# Autodesk Inventor assembly: FRC Fixed Field 2018_sldasm
(part 2 of 2)
- C:\Users\CAD\Documents\GitHub\FIRST Power Up Field CAD\Body_1165_sldprt.ipt
- C:\Users\CAD\Documents\GitHub\FIRST Power Up Field CAD\Body_1166_sldprt.ipt
- C:\Users\CAD\Documents\GitHub\FIRST Power Up Field CAD\Body_1167_sldprt.ipt
- C:\Users\CAD\Documents\GitHub\FIRST Power Up Field CAD\Body_1168_sldprt.ipt
- C:\Users\CAD\Documents\GitHub\FIRST Power Up Field CAD\Body_1169_sldprt.ipt
- C:\Users\CAD\Documents\GitHub\FIRST Power Up Field CAD\Body_1170_sldprt.ipt
- C:\Users\CAD\Documents\GitHub\FIRST Power Up Field CAD\Body_1171_sldprt.ipt
- C:\Users\CAD\Documents\GitHub\FIRST Power Up Field CAD\Body_1172_sldprt.ipt
- C:\Users\CAD\Documents\GitHub\FIRST Power Up Field CAD\Body_1173_sldprt.ipt
- C:\Users\CAD\Documents\GitHub\FIRST Power Up Field CAD\Body_1174_sldprt.ipt
- C:\Users\CAD\Documents\GitHub\FIRST Power Up Field CAD\Body_1175_sldprt.ipt
- C:\Users\CAD\Documents\GitHub\FIRST Power Up Field CAD\Body_1176_sldprt.ipt
- C:\Users\CAD\Documents\GitHub\FIRST Power Up Field CAD\Body_1177_sldprt.ipt
- C:\Users\CAD\Documents\GitHub\FIRST Power Up Field CAD\Body_1178_sldprt.ipt
- C:\Users\CAD\Documents\GitHub\FIRST Power Up Field CAD\Body_1179_sldprt.ipt
- C:\Users\CAD\Documents\GitHub\FIRST Power Up Field CAD\Body_1180_sldprt.ipt
- C:\Users\CAD\Documents\GitHub\FIRST Power Up Field CAD\Body_1181_sldprt.ipt
- C:\Users\CAD\Documents\GitHub\FIRST Power Up Field CAD\Body_1182_sldprt.ipt
- C:\Users\CAD\Documents\GitHub\FIRST Power Up Field CAD\Body_1183_sldprt.ipt
- C:\Users\CAD\Documents\GitHub\FIRST Power Up Field CAD\Body_1184_sldprt.ipt
- C:\Users\CAD\Documents\GitHub\FIRST Power Up Field CAD\Body_1185_sldprt.ipt
- C:\Users\CAD\Documents\GitHub\FIRST Power Up Field CAD\Body_1186_sldprt.ipt
- C:\Users\CAD\Documents\GitHub\FIRST Power Up Field CAD\Body_1187_sldprt.ipt
- C:\Users\CAD\Documents\GitHub\FIRST Power Up Field CAD\Body_1188_sldprt.ipt
- C:\Users\CAD\Documents\GitHub\FIRST Power Up Field CAD\Body_1189_sldprt.ipt
- C:\Users\CAD\Documents\GitHub\FIRST Power Up Field CAD\Body_1190_sldprt.ipt
- C:\Users\CAD\Documents\GitHub\FIRST Power Up Field CAD\Body_1191_sldprt.ipt
- C:\Users\CAD\Documents\GitHub\FIRST Power Up Field CAD\Body_1192_sldprt.ipt
- C:\Users\CAD\Documents\GitHub\FIRST Power Up Field CAD\Body_1193_sldprt.ipt
- C:\Users\CAD\Documents\GitHub\FIRST Power Up Field CAD\Body_1194_sldprt.ipt
- C:\Users\CAD\Documents\GitHub\FIRST Power Up Field CAD\Body_1195_sldprt.ipt
- C:\Users\CAD\Documents\GitHub\FIRST Power Up Field CAD\Body_1196_sldprt.ipt
- C:\Users\CAD\Documents\GitHub\FIRST Power Up Field CAD\Body_1197_sldprt.ipt
- C:\Users\CAD\Documents\GitHub\FIRST Power Up Field CAD\Body_1198_sldprt.ipt
- C:\Users\CAD\Documents\GitHub\FIRST Power Up Field CAD\Body_1199_sldprt.ipt
- C:\Users\CAD\Documents\GitHub\FIRST Power Up Field CAD\Body_1200_sldprt.ipt
- C:\Users\CAD\Documents\GitHub\FIRST Power Up Field CAD\Body_1201_sldprt.ipt
- C:\Users\CAD\Documents\GitHub\FIRST Power Up Field CAD\Body_1202_sldprt.ipt
- C:\Users\CAD\Documents\GitHub\FIRST Power Up Field CAD\Body_1203_sldprt.ipt
- C:\Users\CAD\Documents\GitHub\FIRST Power Up Field CAD\Body_1204_sldprt.ipt
- C:\Users\CAD\Documents\GitHub\FIRST Power Up Field CAD\Body_1205_sldprt.ipt
- C:\Users\CAD\Documents\GitHub\FIRST Power Up Field CAD\Body_1206_sldprt.ipt
- C:\Users\CAD\Documents\GitHub\FIRST Power Up Field CAD\Body_1207_sldprt.ipt
- C:\Users\CAD\Documents\GitHub\FIRST Power Up Field CAD\Body_1208_sldprt.ipt
- C:\Users\CAD\Documents\GitHub\FIRST Power Up Field CAD\Body_1209_sldprt.ipt
- C:\Users\CAD\Documents\GitHub\FIRST Power Up Field CAD\Body_1210_sldprt.ipt
- C:\Users\CAD\Documents\GitHub\FIRST Power Up Field CAD\Body_1211_sldprt.ipt
- C:\Users\CAD\Documents\GitHub\FIRST Power Up Field CAD\Body_1212_sldprt.ipt
- C:\Users\CAD\Documents\GitHub\FIRST Power Up Field CAD\Body_1213_sldprt.ipt
- C:\Users\CAD\Documents\GitHub\FIRST Power Up Field CAD\Body_1214_sldprt.ipt
- C:\Users\CAD\Documents\GitHub\FIRST Power Up Field CAD\Body_1215_sldprt.ipt
- C:\Users\CAD\Documents\GitHub\FIRST Power Up Field CAD\Body_1216_sldprt.ipt
- C:\Users\CAD\Documents\GitHub\FIRST Power Up Field CAD\Body_1217_sldprt.ipt
- C:\Users\CAD\Documents\GitHub\FIRST Power Up Field CAD\Body_1218_sldprt.ipt
- C:\Users\CAD\Documents\GitHub\FIRST Power Up Field CAD\Body_1219_sldprt.ipt
- C:\Users\CAD\Documents\GitHub\FIRST Power Up Field CAD\Body_1220_sldprt.ipt
- C:\Users\CAD\Documents\GitHub\FIRST Power Up Field CAD\Body_1221_sldprt.ipt
- C:\Users\CAD\Documents\GitHub\FIRST Power Up Field CAD\Body_1222_sldprt.ipt
- C:\Users\CAD\Documents\GitHub\FIRST Power Up Field CAD\Body_1223_sldprt.ipt
- C:\Users\CAD\Documents\GitHub\FIRST Power Up Field CAD\Body_1224_sldprt.ipt
- C:\Users\CAD\Documents\GitHub\FIRST Power Up Field CAD\Body_1225_sldprt.ipt
- C:\Users\CAD\Documents\GitHub\FIRST Power Up Field CAD\Body_1226_sldprt.ipt
- C:\Users\CAD\Documents\GitHub\FIRST Power Up Field CAD\Body_1227_sldprt.ipt
- C:\Users\CAD\Documents\GitHub\FIRST Power Up Field CAD\Body_1228_sldprt.ipt
- C:\Users\CAD\Documents\GitHub\FIRST Power Up Field CAD\Body_1229_sldprt.ipt
- C:\Users\CAD\Documents\GitHub\FIRST Power Up Field CAD\Body_1230_sldprt.ipt
- C:\Users\CAD\Documents\GitHub\FIRST Power Up Field CAD\Body_1231_sldprt.ipt
- C:\Users\CAD\Documents\GitHub\FIRST Power Up Field CAD\Body_1232_sldprt.ipt
- C:\Users\CAD\Documents\GitHub\FIRST Power Up Field CAD\Body_1233_sldprt.ipt
- C:\Users\CAD\Documents\GitHub\FIRST Power Up Field CAD\Body_1234_sldprt.ipt
- C:\Users\CAD\Documents\GitHub\FIRST Power Up Field CAD\Body_1235_sldprt.ipt
- C:\Users\CAD\Documents\GitHub\FIRST Power Up Field CAD\Body_1236_sldprt.ipt
- C:\Users\CAD\Documents\GitHub\FIRST Power Up Field CAD\Body_1237_sldprt.ipt
- C:\Users\CAD\Documents\GitHub\FIRST Power Up Field CAD\Body_1238_sldprt.ipt
- C:\Users\CAD\Documents\GitHub\FIRST Power Up Field CAD\Body_1239_sldprt.ipt
- C:\Users\CAD\Documents\GitHub\FIRST Power Up Field CAD\Body_1240_sldprt.ipt
- C:\Users\CAD\Documents\GitHub\FIRST Power Up Field CAD\Body_1241_sldprt.ipt
- C:\Users\CAD\Documents\GitHub\FIRST Power Up Field CAD\Body_1242_sldprt.ipt
- C:\Users\CAD\Documents\GitHub\FIRST Power Up Field CAD\Body_1243_sldprt.ipt
- C:\Users\CAD\Documents\GitHub\FIRST Power Up Field CAD\Body_1244_sldprt.ipt
- C:\Users\CAD\Documents\GitHub\FIRST Power Up Field CAD\Body_1245_sldprt.ipt
- C:\Users\CAD\Documents\GitHub\FIRST Power Up Field CAD\Body_1246_sldprt.ipt
- C:\Users\CAD\Documents\GitHub\FIRST Power Up Field CAD\Body_1247_sldprt.ipt
- C:\Users\CAD\Documents\GitHub\FIRST Power Up Field CAD\Body_1248_sldprt.ipt
- C:\Users\CAD\Documents\GitHub\FIRST Power Up Field CAD\Body_1249_sldprt.ipt
- C:\Users\CAD\Documents\GitHub\FIRST Power Up Field CAD\Body_1250_sldprt.ipt
- C:\Users\CAD\Documents\GitHub\FIRST Power Up Field CAD\Body_1251_sldprt.ipt
- C:\Users\CAD\Documents\GitHub\FIRST Power Up Field CAD\Body_1252_sldprt.ipt
- C:\Users\CAD\Documents\GitHub\FIRST Power Up Field CAD\Body_1253_sldprt.ipt
- C:\Users\CAD\Documents\GitHub\FIRST Power Up Field CAD\Body_1254_sldprt.ipt
- C:\Users\CAD\Documents\GitHub\FIRST Power Up Field CAD\Body_1255_sldprt.ipt
- C:\Users\CAD\Documents\GitHub\FIRST Power Up Field CAD\Body_1256_sldprt.ipt
- C:\Users\CAD\Documents\GitHub\FIRST Power Up Field CAD\Body_1257_sldprt.ipt
- C:\Users\CAD\Documents\GitHub\FIRST Power Up Field CAD\Body_1258_sldprt.ipt
- C:\Users\CAD\Documents\GitHub\FIRST Power Up Field CAD\Body_1259_sldprt.ipt
- C:\Users\CAD\Documents\GitHub\FIRST Power Up Field CAD\Body_1260_sldprt.ipt
- C:\Users\CAD\Documents\GitHub\FIRST Power Up Field CAD\Body_1261_sldprt.ipt
- C:\Users\CAD\Documents\GitHub\FIRST Power Up Field CAD\Body_1262_sldprt.ipt
- C:\Users\CAD\Documents\GitHub\FIRST Power Up Field CAD\Body_1263_sldprt.ipt
- C:\Users\CAD\Documents\GitHub\FIRST Power Up Field CAD\Body_1264_sldprt.ipt
- C:\Users\CAD\Documents\GitHub\FIRST Power Up Field CAD\Body_1265_sldprt.ipt
- C:\Users\CAD\Documents\GitHub\FIRST Power Up Field CAD\Body_1266_sldprt.ipt
- C:\Users\CAD\Documents\GitHub\FIRST Power Up Field CAD\Body_1267_sldprt.ipt
- C:\Users\CAD\Documents\GitHub\FIRST Power Up Field CAD\Body_1268_sldprt.ipt
- C:\Users\CAD\Documents\GitHub\FIRST Power Up Field CAD\Body_1269_sldprt.ipt
- C:\Users\CAD\Documents\GitHub\FIRST Power Up Field CAD\Body_1270_sldprt.ipt
- C:\Users\CAD\Documents\GitHub\FIRST Power Up Field CAD\Body_1271_sldprt.ipt
- C:\Users\CAD\Documents\GitHub\FIRST Power Up Field CAD\Body_1272_sldprt.ipt
- C:\Users\CAD\Documents\GitHub\FIRST Power Up Field CAD\Body_1273_sldprt.ipt
- C:\Users\CAD\Documents\GitHub\FIRST Power Up Field CAD\Body_1274_sldprt.ipt
- C:\Users\CAD\Documents\GitHub\FIRST Power Up Field CAD\Body_1275_sldprt.ipt
- C:\Users\CAD\Documents\GitHub\FIRST Power Up Field CAD\Body_1276_sldprt.ipt
- C:\Users\CAD\Documents\GitHub\FIRST Power Up Field CAD\Body_1277_sldprt.ipt
- C:\Users\CAD\Documents\GitHub\FIRST Power Up Field CAD\Body_1278_sldprt.ipt
- C:\Users\CAD\Documents\GitHub\FIRST Power Up Field CAD\Body_1279_sldprt.ipt
- C:\Users\CAD\Documents\GitHub\FIRST Power Up Field CAD\Body_1280_sldprt.ipt
- C:\Users\CAD\Documents\GitHub\FIRST Power Up Field CAD\Body_1281_sldprt.ipt
- C:\Users\CAD\Documents\GitHub\FIRST Power Up Field CAD\Body_1282_sldprt.ipt
- C:\Users\CAD\Documents\GitHub\FIRST Power Up Field CAD\Body_1283_sldprt.ipt
- C:\Users\CAD\Documents\GitHub\FIRST Power Up Field CAD\Body_1284_sldprt.ipt
- C:\Users\CAD\Documents\GitHub\FIRST Power Up Field CAD\Body_1285_sldprt.ipt
- C:\Users\CAD\Documents\GitHub\FIRST Power Up Field CAD\Body_1286_sldprt.ipt
- C:\Users\CAD\Documents\GitHub\FIRST Power Up Field CAD\Body_1287_sldprt.ipt
- C:\Users\CAD\Documents\GitHub\FIRST Power Up Field CAD\Body_1288_sldprt.ipt
- C:\Users\CAD\Documents\GitHub\FIRST Power Up Field CAD\Body_1289_sldprt.ipt
- C:\Users\CAD\Documents\GitHub\FIRST Power Up Field CAD\Body_1290_sldprt.ipt
- C:\Users\CAD\Documents\GitHub\FIRST Power Up Field CAD\Body_1291_sldprt.ipt
- C:\Users\CAD\Documents\GitHub\FIRST Power Up Field CAD\Body_1292_sldprt.ipt
- C:\Users\CAD\Documents\GitHub\FIRST Power Up Field CAD\Body_1293_sldprt.ipt
- C:\Users\CAD\Documents\GitHub\FIRST Power Up Field CAD\Body_1294_sldprt.ipt
- C:\Users\CAD\Documents\GitHub\FIRST Power Up Field CAD\Body_1295_sldprt.ipt
- C:\Users\CAD\Documents\GitHub\FIRST Power Up Field CAD\Body_1296_sldprt.ipt
- C:\Users\CAD\Documents\GitHub\FIRST Power Up Field CAD\Body_1297_sldprt.ipt
- C:\Users\CAD\Documents\GitHub\FIRST Power Up Field CAD\Body_1298_sldprt.ipt
- C:\Users\CAD\Documents\GitHub\FIRST Power Up Field CAD\Body_1299_sldprt.ipt
- C:\Users\CAD\Documents\GitHub\FIRST Power Up Field CAD\Body_1300_sldprt.ipt
- C:\Users\CAD\Documents\GitHub\FIRST Power Up Field CAD\Body_1301_sldprt.ipt
- C:\Users\CAD\Documents\GitHub\FIRST Power Up Field CAD\Body_1302_sldprt.ipt
- C:\Users\CAD\Documents\GitHub\FIRST Power Up Field CAD\Body_1303_sldprt.ipt
- C:\Users\CAD\Documents\GitHub\FIRST Power Up Field CAD\Body_1304_sldprt.ipt
- C:\Users\CAD\Documents\GitHub\FIRST Power Up Field CAD\Body_1305_sldprt.ipt
- C:\Users\CAD\Documents\GitHub\FIRST Power Up Field CAD\Body_1306_sldprt.ipt
- C:\Users\CAD\Documents\GitHub\FIRST Power Up Field CAD\Body_1307_sldprt.ipt
- C:\Users\CAD\Documents\GitHub\FIRST Power Up Field CAD\Body_1308_sldprt.ipt
- C:\Users\CAD\Documents\GitHub\FIRST Power Up Field CAD\Body_1309_sldprt.ipt
- C:\Users\CAD\Documents\GitHub\FIRST Power Up Field CAD\Body_1310_sldprt.ipt
- C:\Users\CAD\Documents\GitHub\FIRST Power Up Field CAD\Body_1311_sldprt.ipt
- C:\Users\CAD\Documents\GitHub\FIRST Power Up Field CAD\Body_1312_sldprt.ipt
- C:\Users\CAD\Documents\GitHub\FIRST Power Up Field CAD\Body_1313_sldprt.ipt
- C:\Users\CAD\Documents\GitHub\FIRST Power Up Field CAD\Body_1314_sldprt.ipt
- C:\Users\CAD\Documents\GitHub\FIRST Power Up Field CAD\Body_1315_sldprt.ipt
- C:\Users\CAD\Documents\GitHub\FIRST Power Up Field CAD\Body_1316_sldprt.ipt
- C:\Users\CAD\Documents\GitHub\FIRST Power Up Field CAD\Body_1317_sldprt.ipt
- C:\Users\CAD\Documents\GitHub\FIRST Power Up Field CAD\Body_1318_sldprt.ipt
- C:\Users\CAD\Documents\GitHub\FIRST Power Up Field CAD\Body_1319_sldprt.ipt
- C:\Users\CAD\Documents\GitHub\FIRST Power Up Field CAD\Body_1320_sldprt.ipt
- C:\Users\CAD\Documents\GitHub\FIRST Power Up Field CAD\Body_1321_sldprt.ipt
- C:\Users\CAD\Documents\GitHub\FIRST Power Up Field CAD\Body_1322_sldprt.ipt
- C:\Users\CAD\Documents\GitHub\FIRST Power Up Field CAD\Body_1323_sldprt.ipt
- C:\Users\CAD\Documents\GitHub\FIRST Power Up Field CAD\Body_1324_sldprt.ipt
- C:\Users\CAD\Documents\GitHub\FIRST Power Up Field CAD\Body_1325_sldprt.ipt
- C:\Users\CAD\Documents\GitHub\FIRST Power Up Field CAD\Body_1326_sldprt.ipt
- C:\Users\CAD\Documents\GitHub\FIRST Power Up Field CAD\Body_1327_sldprt.ipt
- C:\Users\CAD\Documents\GitHub\FIRST Power Up Field CAD\Body_1328_sldprt.ipt
- C:\Users\CAD\Documents\GitHub\FIRST Power Up Field CAD\Body_1329_sldprt.ipt
- C:\Users\CAD\Documents\GitHub\FIRST Power Up Field CAD\Body_1330_sldprt.ipt
- C:\Users\CAD\Documents\GitHub\FIRST Power Up Field CAD\Body_1331_sldprt.ipt
- C:\Users\CAD\Documents\GitHub\FIRST Power Up Field CAD\Body_1332_sldprt.ipt
- C:\Users\CAD\Documents\GitHub\FIRST Power Up Field CAD\Body_1333_sldprt.ipt
- C:\Users\CAD\Documents\GitHub\FIRST Power Up Field CAD\Body_1334_sldprt.ipt
- C:\Users\CAD\Documents\GitHub\FIRST Power Up Field CAD\Body_1335_sldprt.ipt
- C:\Users\CAD\Documents\GitHub\FIRST Power Up Field CAD\Body_1336_sldprt.ipt
- C:\Users\CAD\Documents\GitHub\FIRST Power Up Field CAD\Body_1337_sldprt.ipt
- C:\Users\CAD\Documents\GitHub\FIRST Power Up Field CAD\Body_1338_sldprt.ipt
- C:\Users\CAD\Documents\GitHub\FIRST Power Up Field CAD\Body_1339_sldprt.ipt
- C:\Users\CAD\Documents\GitHub\FIRST Power Up Field CAD\Body_1340_sldprt.ipt
- C:\Users\CAD\Documents\GitHub\FIRST Power Up Field CAD\Body_1341_sldprt.ipt
- C:\Users\CAD\Documents\GitHub\FIRST Power Up Field CAD\Body_1342_sldprt.ipt
- C:\Users\CAD\Documents\GitHub\FIRST Power Up Field CAD\Body_1343_sldprt.ipt
- C:\Users\CAD\Documents\GitHub\FIRST Power Up Field CAD\Body_1344_sldprt.ipt
- C:\Users\CAD\Documents\GitHub\FIRST Power Up Field CAD\Body_1345_sldprt.ipt
- C:\Users\CAD\Documents\GitHub\FIRST Power Up Field CAD\Body_1346_sldprt.ipt
- C:\Users\CAD\Documents\GitHub\FIRST Power Up Field CAD\Body_1347_sldprt.ipt
- C:\Users\CAD\Documents\GitHub\FIRST Power Up Field CAD\Body_1348_sldprt.ipt
- C:\Users\CAD\Documents\GitHub\FIRST Power Up Field CAD\Body_1349_sldprt.ipt
- C:\Users\CAD\Documents\GitHub\FIRST Power Up Field CAD\Body_1350_sldprt.ipt
- C:\Users\CAD\Documents\GitHub\FIRST Power Up Field CAD\Body_1351_sldprt.ipt
- C:\Users\CAD\Documents\GitHub\FIRST Power Up Field CAD\Body_1352_sldprt.ipt
- C:\Users\CAD\Documents\GitHub\FIRST Power Up Field CAD\Body_1353_sldprt.ipt
- C:\Users\CAD\Documents\GitHub\FIRST Power Up Field CAD\Body_1354_sldprt.ipt
- C:\Users\CAD\Documents\GitHub\FIRST Power Up Field CAD\Body_1355_sldprt.ipt
- C:\Users\CAD\Documents\GitHub\FIRST Power Up Field CAD\Body_1356_sldprt.ipt
- C:\Users\CAD\Documents\GitHub\FIRST Power Up Field CAD\Body_1357_sldprt.ipt
- C:\Users\CAD\Documents\GitHub\FIRST Power Up Field CAD\Body_1358_sldprt.ipt
- C:\Users\CAD\Documents\GitHub\FIRST Power Up Field CAD\Body_1359_sldprt.ipt
- C:\Users\CAD\Documents\GitHub\FIRST Power Up Field CAD\Body_1360_sldprt.ipt
- C:\Users\CAD\Documents\GitHub\FIRST Power Up Field CAD\Body_1361_sldprt.ipt
- C:\Users\CAD\Documents\GitHub\FIRST Power Up Field CAD\Body_1362_sldprt.ipt
- C:\Users\CAD\Documents\GitHub\FIRST Power Up Field CAD\Body_1363_sldprt.ipt
- C:\Users\CAD\Documents\GitHub\FIRST Power Up Field CAD\Body_1364_sldprt.ipt
- C:\Users\CAD\Documents\GitHub\FIRST Power Up Field CAD\Body_1365_sldprt.ipt
- C:\Users\CAD\Documents\GitHub\FIRST Power Up Field CAD\Body_1366_sldprt.ipt
- C:\Users\CAD\Documents\GitHub\FIRST Power Up Field CAD\Body_1367_sldprt.ipt
- C:\Users\CAD\Documents\GitHub\FIRST Power Up Field CAD\Body_1368_sldprt.ipt
- C:\Users\CAD\Documents\GitHub\FIRST Power Up Field CAD\Body_1369_sldprt.ipt
- C:\Users\CAD\Documents\GitHub\FIRST Power Up Field CAD\Body_1370_sldprt.ipt
- C:\Users\CAD\Documents\GitHub\FIRST Power Up Field CAD\Body_1371_sldprt.ipt
- C:\Users\CAD\Documents\GitHub\FIRST Power Up Field CAD\Body_1372_sldprt.ipt
- C:\Users\CAD\Documents\GitHub\FIRST Power Up Field CAD\Body_1373_sldprt.ipt
- C:\Users\CAD\Documents\GitHub\FIRST Power Up Field CAD\Body_1374_sldprt.ipt
- C:\Users\CAD\Documents\GitHub\FIRST Power Up Field CAD\Body_1375_sldprt.ipt
- C:\Users\CAD\Documents\GitHub\FIRST Power Up Field CAD\Body_1376_sldprt.ipt
- C:\Users\CAD\Documents\GitHub\FIRST Power Up Field CAD\Body_1377_sldprt.ipt
- C:\Users\CAD\Documents\GitHub\FIRST Power Up Field CAD\Body_1378_sldprt.ipt
- C:\Users\CAD\Documents\GitHub\FIRST Power Up Field CAD\Body_1379_sldprt.ipt
- C:\Users\CAD\Documents\GitHub\FIRST Power Up Field CAD\Body_1380_sldprt.ipt
- C:\Users\CAD\Documents\GitHub\FIRST Power Up Field CAD\Body_1381_sldprt.ipt
- C:\Users\CAD\Documents\GitHub\FIRST Power Up Field CAD\Body_1382_sldprt.ipt
- C:\Users\CAD\Documents\GitHub\FIRST Power Up Field CAD\Body_1383_sldprt.ipt
- C:\Users\CAD\Documents\GitHub\FIRST Power Up Field CAD\Body_1384_sldprt.ipt
- C:\Users\CAD\Documents\GitHub\FIRST Power Up Field CAD\Body_1385_sldprt.ipt
- C:\Users\CAD\Documents\GitHub\FIRST Power Up Field CAD\Body_1386_sldprt.ipt
- C:\Users\CAD\Documents\GitHub\FIRST Power Up Field CAD\Body_1387_sldprt.ipt
- C:\Users\CAD\Documents\GitHub\FIRST Power Up Field CAD\Body_1388_sldprt.ipt
- C:\Users\CAD\Documents\GitHub\FIRST Power Up Field CAD\Body_1389_sldprt.ipt
- C:\Users\CAD\Documents\GitHub\FIRST Power Up Field CAD\Body_1390_sldprt.ipt
- C:\Users\CAD\Documents\GitHub\FIRST Power Up Field CAD\Body_1391_sldprt.ipt
- C:\Users\CAD\Documents\GitHub\FIRST Power Up Field CAD\Body_1392_sldprt.ipt
- C:\Users\CAD\Documents\GitHub\FIRST Power Up Field CAD\Body_1393_sldprt.ipt
- C:\Users\CAD\Documents\GitHub\FIRST Power Up Field CAD\Body_1394_sldprt.ipt
- C:\Users\CAD\Documents\GitHub\FIRST Power Up Field CAD\Body_1395_sldprt.ipt
- C:\Users\CAD\Documents\GitHub\FIRST Power Up Field CAD\Body_1396_sldprt.ipt
- C:\Users\CAD\Documents\GitHub\FIRST Power Up Field CAD\Body_1397_sldprt.ipt
- C:\Users\CAD\Documents\GitHub\FIRST Power Up Field CAD\Body_1398_sldprt.ipt
- C:\Users\CAD\Documents\GitHub\FIRST Power Up Field CAD\Body_1399_sldprt.ipt
- C:\Users\CAD\Documents\GitHub\FIRST Power Up Field CAD\Body_1400_sldprt.ipt
- C:\Users\CAD\Documents\GitHub\FIRST Power Up Field CAD\Body_1401_sldprt.ipt
- C:\Users\CAD\Documents\GitHub\FIRST Power Up Field CAD\Body_1402_sldprt.ipt
- C:\Users\CAD\Documents\GitHub\FIRST Power Up Field CAD\Body_1403_sldprt.ipt
- C:\Users\CAD\Documents\GitHub\FIRST Power Up Field CAD\Body_1404_sldprt.ipt
- C:\Users\CAD\Documents\GitHub\FIRST Power Up Field CAD\Body_1405_sldprt.ipt
- C:\Users\CAD\Documents\GitHub\FIRST Power Up Field CAD\Body_1406_sldprt.ipt
- C:\Users\CAD\Documents\GitHub\FIRST Power Up Field CAD\Body_1407_sldprt.ipt
- C:\Users\CAD\Documents\GitHub\FIRST Power Up Field CAD\Body_1408_sldprt.ipt
- C:\Users\CAD\Documents\GitHub\FIRST Power Up Field CAD\Body_1409_sldprt.ipt
- C:\Users\CAD\Documents\GitHub\FIRST Power Up Field CAD\Body_1410_sldprt.ipt
- C:\Users\CAD\Documents\GitHub\FIRST Power Up Field CAD\Body_1411_sldprt.ipt
- C:\Users\CAD\Documents\GitHub\FIRST Power Up Field CAD\Body_1412_sldprt.ipt
- C:\Users\CAD\Documents\GitHub\FIRST Power Up Field CAD\Body_1413_sldprt.ipt
- C:\Users\CAD\Documents\GitHub\FIRST Power Up Field CAD\Body_1414_sldprt.ipt
- C:\Users\CAD\Documents\GitHub\FIRST Power Up Field CAD\Body_1415_sldprt.ipt
- C:\Users\CAD\Documents\GitHub\FIRST Power Up Field CAD\Body_1416_sldprt.ipt
- C:\Users\CAD\Documents\GitHub\FIRST Power Up Field CAD\Body_1417_sldprt.ipt
- C:\Users\CAD\Documents\GitHub\FIRST Power Up Field CAD\Body_1418_sldprt.ipt
- C:\Users\CAD\Documents\GitHub\FIRST Power Up Field CAD\Body_1419_sldprt.ipt
- C:\Users\CAD\Documents\GitHub\FIRST Power Up Field CAD\Body_1420_sldprt.ipt
- C:\Users\CAD\Documents\GitHub\FIRST Power Up Field CAD\Body_1421_sldprt.ipt
- C:\Users\CAD\Documents\GitHub\FIRST Power Up Field CAD\Body_1422_sldprt.ipt
- C:\Users\CAD\Documents\GitHub\FIRST Power Up Field CAD\Body_1423_sldprt.ipt
- C:\Users\CAD\Documents\GitHub\FIRST Power Up Field CAD\Body_1424_sldprt.ipt
- C:\Users\CAD\Documents\GitHub\FIRST Power Up Field CAD\Body_1425_sldprt.ipt
- C:\Users\CAD\Documents\GitHub\FIRST Power Up Field CAD\Body_1426_sldprt.ipt
- C:\Users\CAD\Documents\GitHub\FIRST Power Up Field CAD\Body_1427_sldprt.ipt
- C:\Users\CAD\Documents\GitHub\FIRST Power Up Field CAD\Body_1428_sldprt.ipt
- C:\Users\CAD\Documents\GitHub\FIRST Power Up Field CAD\Body_1429_sldprt.ipt
- C:\Users\CAD\Documents\GitHub\FIRST Power Up Field CAD\Body_1430_sldprt.ipt
- C:\Users\CAD\Documents\GitHub\FIRST Power Up Field CAD\Body_1431_sldprt.ipt
- C:\Users\CAD\Documents\GitHub\FIRST Power Up Field CAD\Body_1432_sldprt.ipt
- C:\Users\CAD\Documents\GitHub\FIRST Power Up Field CAD\Body_1433_sldprt.ipt
- C:\Users\CAD\Documents\GitHub\FIRST Power Up Field CAD\Body_1434_sldprt.ipt
- C:\Users\CAD\Documents\GitHub\FIRST Power Up Field CAD\Body_1435_sldprt.ipt
- C:\Users\CAD\Documents\GitHub\FIRST Power Up Field CAD\Body_1436_sldprt.ipt
- C:\Users\CAD\Documents\GitHub\FIRST Power Up Field CAD\Body_1437_sldprt.ipt
- C:\Users\CAD\Documents\GitHub\FIRST Power Up Field CAD\Body_1438_sldprt.ipt
- C:\Users\CAD\Documents\GitHub\FIRST Power Up Field CAD\Body_1439_sldprt.ipt
- C:\Users\CAD\Documents\GitHub\FIRST Power Up Field CAD\Body_1440_sldprt.ipt
- C:\Users\CAD\Documents\GitHub\FIRST Power Up Field CAD\Body_1441_sldprt.ipt
- C:\Users\CAD\Documents\GitHub\FIRST Power Up Field CAD\Body_1442_sldprt.ipt
- C:\Users\CAD\Documents\GitHub\FIRST Power Up Field CAD\Body_1443_sldprt.ipt
- C:\Users\CAD\Documents\GitHub\FIRST Power Up Field CAD\Body_1444_sldprt.ipt
- C:\Users\CAD\Documents\GitHub\FIRST Power Up Field CAD\Body_1445_sldprt.ipt
- C:\Users\CAD\Documents\GitHub\FIRST Power Up Field CAD\Body_1446_sldprt.ipt
- C:\Users\CAD\Documents\GitHub\FIRST Power Up Field CAD\Body_1447_sldprt.ipt
- C:\Users\CAD\Documents\GitHub\FIRST Power Up Field CAD\Body_1448_sldprt.ipt
- C:\Users\CAD\Documents\GitHub\FIRST Power Up Field CAD\Body_1449_sldprt.ipt
- C:\Users\CAD\Documents\GitHub\FIRST Power Up Field CAD\Body_1450_sldprt.ipt
- C:\Users\CAD\Documents\GitHub\FIRST Power Up Field CAD\Body_1451_sldprt.ipt
- C:\Users\CAD\Documents\GitHub\FIRST Power Up Field CAD\Body_1452_sldprt.ipt
- C:\Users\CAD\Documents\GitHub\FIRST Power Up Field CAD\Body_1453_sldprt.ipt
- C:\Users\CAD\Documents\GitHub\FIRST Power Up Field CAD\Body_1454_sldprt.ipt
- C:\Users\CAD\Documents\GitHub\FIRST Power Up Field CAD\Body_1455_sldprt.ipt
- C:\Users\CAD\Documents\GitHub\FIRST Power Up Field CAD\Body_1456_sldprt.ipt
- C:\Users\CAD\Documents\GitHub\FIRST Power Up Field CAD\Body_1457_sldprt.ipt
- C:\Users\CAD\Documents\GitHub\FIRST Power Up Field CAD\Body_1458_sldprt.ipt
- C:\Users\CAD\Documents\GitHub\FIRST Power Up Field CAD\Body_1459_sldprt.ipt
- C:\Users\CAD\Documents\GitHub\FIRST Power Up Field CAD\Body_1460_sldprt.ipt
- C:\Users\CAD\Documents\GitHub\FIRST Power Up Field CAD\Body_1461_sldprt.ipt
- C:\Users\CAD\Documents\GitHub\FIRST Power Up Field CAD\Body_1462_sldprt.ipt
- C:\Users\CAD\Documents\GitHub\FIRST Power Up Field CAD\Body_1463_sldprt.ipt
- C:\Users\CAD\Documents\GitHub\FIRST Power Up Field CAD\Body_1464_sldprt.ipt
- C:\Users\CAD\Documents\GitHub\FIRST Power Up Field CAD\Body_1465_sldprt.ipt
- C:\Users\CAD\Documents\GitHub\FIRST Power Up Field CAD\Body_1466_sldprt.ipt
## Components (942 placed, 942 different names)
1. Body_525_sldprt_1001
2. Body_526_sldprt_1002
3. Body_527_sldprt_1003
4. Body_528_sldprt_1004
5. Body_529_sldprt_1005
6. Body_530_sldprt_1006
7. Body_531_sldprt_1007
8. Body_532_sldprt_1008
9. Body_533_sldprt_1009
10. Body_534_sldprt_1010
11. Body_535_sldprt_1011
12. Body_536_sldprt_1012
13. Body_537_sldprt_1013
14. Body_538_sldprt_1014
15. Body_539_sldprt_1015
16. Body_540_sldprt_1016
17. Body_541_sldprt_1017
18. Body_542_sldprt_1018
19. Body_543_sldprt_1019
20. Body_544_sldprt_1020
21. Body_545_sldprt_1021
22. Body_546_sldprt_1022
23. Body_547_sldprt_1023
24. Body_548_sldprt_1024
25. Body_549_sldprt_1025
26. Body_550_sldprt_1026
27. Body_551_sldprt_1027
28. Body_552_sldprt_1028
29. Body_553_sldprt_1029
30. Body_554_sldprt_1030
31. Body_555_sldprt_1031
32. Body_556_sldprt_1032
33. Body_557_sldprt_1033
34. Body_558_sldprt_1034
35. Body_559_sldprt_1035
36. Body_560_sldprt_1036
37. Body_561_sldprt_1037
38. Body_562_sldprt_1038
39. Body_563_sldprt_1039
40. Body_564_sldprt_1040
41. Body_565_sldprt_1041
42. Body_566_sldprt_1042
43. Body_567_sldprt_1043
44. Body_568_sldprt_1044
45. Body_569_sldprt_1045
46. Body_570_sldprt_1046
47. Body_571_sldprt_1047
48. Body_572_sldprt_1048
49. Body_573_sldprt_1049
50. Body_574_sldprt_1050
51. Body_575_sldprt_1051
52. Body_576_sldprt_1052
53. Body_577_sldprt_1053
54. Body_578_sldprt_1054
55. Body_579_sldprt_1055
56. Body_580_sldprt_1056
57. Body_581_sldprt_1057
58. Body_582_sldprt_1058
59. Body_583_sldprt_1059
60. Body_584_sldprt_1060
61. Body_585_sldprt_1061
62. Body_586_sldprt_1062
63. Body_587_sldprt_1063
64. Body_588_sldprt_1064
65. Body_589_sldprt_1065
66. Body_590_sldprt_1066
67. Body_591_sldprt_1067
68. Body_592_sldprt_1068
69. Body_593_sldprt_1069
70. Body_594_sldprt_1070
71. Body_595_sldprt_1071
72. Body_596_sldprt_1072
73. Body_597_sldprt_1073
74. Body_598_sldprt_1074
75. Body_599_sldprt_1075
76. Body_600_sldprt_1076
77. Body_601_sldprt_1077
78. Body_602_sldprt_1078
79. Body_603_sldprt_1079
80. Body_604_sldprt_1080
81. Body_605_sldprt_1081
82. Body_606_sldprt_1082
83. Body_607_sldprt_1083
84. Body_608_sldprt_1084
85. Body_609_sldprt_1085
86. Body_610_sldprt_1086
87. Body_611_sldprt_1087
88. Body_612_sldprt_1088
89. Body_613_sldprt_1089
90. Body_614_sldprt_1090
91. Body_615_sldprt_1091
92. Body_616_sldprt_1092
93. Body_617_sldprt_1093
94. Body_618_sldprt_1094
95. Body_619_sldprt_1095
96. Body_620_sldprt_1096
97. Body_621_sldprt_1097
98. Body_622_sldprt_1098
99. Body_623_sldprt_1099
100. Body_624_sldprt_1100
101. Body_625_sldprt_1101
102. Body_626_sldprt_1102
103. Body_627_sldprt_1103
104. Body_628_sldprt_1104
105. Body_629_sldprt_1105
106. Body_630_sldprt_1106
107. Body_631_sldprt_1107
108. Body_632_sldprt_1108
109. Body_633_sldprt_1109
110. Body_634_sldprt_1110
111. Body_635_sldprt_1111
112. Body_636_sldprt_1112
113. Body_637_sldprt_1113
114. Body_638_sldprt_1114
115. Body_639_sldprt_1115
116. Body_640_sldprt_1116
117. Body_641_sldprt_1117
118. Body_642_sldprt_1118
119. Body_643_sldprt_1119
120. Body_644_sldprt_1120
121. Body_645_sldprt_1121
122. Body_646_sldprt_1122
123. Body_647_sldprt_1123
124. Body_648_sldprt_1124
125. Body_649_sldprt_1125
126. Body_650_sldprt_1126
127. Body_651_sldprt_1127
128. Body_652_sldprt_1128
129. Body_653_sldprt_1129
130. Body_654_sldprt_1130
131. Body_655_sldprt_1131
132. Body_656_sldprt_1132
133. Body_657_sldprt_1133
134. Body_658_sldprt_1134
135. Body_659_sldprt_1135
136. Body_660_sldprt_1136
137. Body_661_sldprt_1137
138. Body_662_sldprt_1138
139. Body_663_sldprt_1139
140. Body_664_sldprt_1140
141. Body_665_sldprt_1141
142. Body_666_sldprt_1142
143. Body_667_sldprt_1143
144. Body_668_sldprt_1144
145. Body_669_sldprt_1145
146. Body_670_sldprt_1146
147. Body_671_sldprt_1147
148. Body_672_sldprt_1148
149. Body_673_sldprt_1149
150. Body_674_sldprt_1150
151. Body_675_sldprt_1151
152. Body_676_sldprt_1152
153. Body_677_sldprt_1153
154. Body_678_sldprt_1154
155. Body_679_sldprt_1155
156. Body_680_sldprt_1156
157. Body_681_sldprt_1157
158. Body_682_sldprt_1158
159. Body_683_sldprt_1159
160. Body_684_sldprt_1160
161. Body_685_sldprt_1161
162. Body_686_sldprt_1162
163. Body_687_sldprt_1163
164. Body_688_sldprt_1164
165. Body_689_sldprt_1165
166. Body_690_sldprt_1166
167. Body_691_sldprt_1167
168. Body_692_sldprt_1168
169. Body_693_sldprt_1169
170. Body_694_sldprt_1170
171. Body_695_sldprt_1171
172. Body_696_sldprt_1172
173. Body_697_sldprt_1173
174. Body_698_sldprt_1174
175. Body_699_sldprt_1175
176. Body_700_sldprt_1176
177. Body_701_sldprt_1177
178. Body_702_sldprt_1178
179. Body_703_sldprt_1179
180. Body_704_sldprt_1180
181. Body_705_sldprt_1181
182. Body_706_sldprt_1182
183. Body_707_sldprt_1183
184. Body_708_sldprt_1184
185. Body_709_sldprt_1185
186. Body_710_sldprt_1186
187. Body_711_sldprt_1187
188. Body_712_sldprt_1188
189. Body_713_sldprt_1189
190. Body_714_sldprt_1190
191. Body_715_sldprt_1191
192. Body_716_sldprt_1192
193. Body_717_sldprt_1193
194. Body_718_sldprt_1194
195. Body_719_sldprt_1195
196. Body_720_sldprt_1196
197. Body_721_sldprt_1197
198. Body_722_sldprt_1198
199. Body_723_sldprt_1199
200. Body_724_sldprt_1200
201. Body_725_sldprt_1201
202. Body_726_sldprt_1202
203. Body_727_sldprt_1203
204. Body_728_sldprt_1204
205. Body_729_sldprt_1205
206. Body_730_sldprt_1206
207. Body_731_sldprt_1207
208. Body_732_sldprt_1208
209. Body_733_sldprt_1209
210. Body_734_sldprt_1210
211. Body_735_sldprt_1211
212. Body_736_sldprt_1212
213. Body_737_sldprt_1213
214. Body_738_sldprt_1214
215. Body_739_sldprt_1215
216. Body_740_sldprt_1216
217. Body_741_sldprt_1217
218. Body_742_sldprt_1218
219. Body_743_sldprt_1219
220. Body_744_sldprt_1220
221. Body_745_sldprt_1221
222. Body_746_sldprt_1222
223. Body_747_sldprt_1223
224. Body_748_sldprt_1224
225. Body_749_sldprt_1225
226. Body_750_sldprt_1226
227. Body_751_sldprt_1227
228. Body_752_sldprt_1228
229. Body_753_sldprt_1229
230. Body_754_sldprt_1230
231. Body_755_sldprt_1231
232. Body_756_sldprt_1232
233. Body_757_sldprt_1233
234. Body_758_sldprt_1234
235. Body_759_sldprt_1235
236. Body_760_sldprt_1236
237. Body_761_sldprt_1237
238. Body_762_sldprt_1238
239. Body_763_sldprt_1239
240. Body_764_sldprt_1240
241. Body_765_sldprt_1241
242. Body_766_sldprt_1242
243. Body_767_sldprt_1243
244. Body_768_sldprt_1244
245. Body_769_sldprt_1245
246. Body_770_sldprt_1246
247. Body_771_sldprt_1247
248. Body_772_sldprt_1248
249. Body_773_sldprt_1249
250. Body_774_sldprt_1250
251. Body_775_sldprt_1251
252. Body_776_sldprt_1252
253. Body_777_sldprt_1253
254. Body_778_sldprt_1254
255. Body_779_sldprt_1255
256. Body_780_sldprt_1256
257. Body_781_sldprt_1257
258. Body_782_sldprt_1258
259. Body_783_sldprt_1259
260. Body_784_sldprt_1260
261. Body_785_sldprt_1261
262. Body_786_sldprt_1262
263. Body_787_sldprt_1263
264. Body_788_sldprt_1264
265. Body_789_sldprt_1265
266. Body_790_sldprt_1266
267. Body_791_sldprt_1267
268. Body_792_sldprt_1268
269. Body_793_sldprt_1269
270. Body_794_sldprt_1270
271. Body_795_sldprt_1271
272. Body_796_sldprt_1272
273. Body_797_sldprt_1273
274. Body_798_sldprt_1274
275. Body_799_sldprt_1275
276. Body_800_sldprt_1276
277. Body_801_sldprt_1277
278. Body_802_sldprt_1278
279. Body_803_sldprt_1279
280. Body_804_sldprt_1280
281. Body_805_sldprt_1281
282. Body_806_sldprt_1282
283. Body_807_sldprt_1283
284. Body_808_sldprt_1284
285. Body_809_sldprt_1285
286. Body_810_sldprt_1286
287. Body_811_sldprt_1287
288. Body_812_sldprt_1288
289. Body_813_sldprt_1289
290. Body_814_sldprt_1290
291. Body_815_sldprt_1291
292. Body_816_sldprt_1292
293. Body_817_sldprt_1293
294. Body_818_sldprt_1294
295. Body_819_sldprt_1295
296. Body_820_sldprt_1296
297. Body_821_sldprt_1297
298. Body_822_sldprt_1298
299. Body_823_sldprt_1299
300. Body_824_sldprt_1300
301. Body_825_sldprt_1301
302. Body_826_sldprt_1302
303. Body_827_sldprt_1303
304. Body_828_sldprt_1304
305. Body_829_sldprt_1305
306. Body_830_sldprt_1306
307. Body_831_sldprt_1307
308. Body_832_sldprt_1308
309. Body_833_sldprt_1309
310. Body_834_sldprt_1310
311. Body_835_sldprt_1311
312. Body_836_sldprt_1312
313. Body_837_sldprt_1313
314. Body_838_sldprt_1314
315. Body_839_sldprt_1315
316. Body_840_sldprt_1316
317. Body_841_sldprt_1317
318. Body_842_sldprt_1318
319. Body_843_sldprt_1319
320. Body_844_sldprt_1320
321. Body_845_sldprt_1321
322. Body_846_sldprt_1322
323. Body_847_sldprt_1323
324. Body_848_sldprt_1324
325. Body_849_sldprt_1325
326. Body_850_sldprt_1326
327. Body_851_sldprt_1327
328. Body_852_sldprt_1328
329. Body_853_sldprt_1329
330. Body_854_sldprt_1330
331. Body_855_sldprt_1331
332. Body_856_sldprt_1332
333. Body_857_sldprt_1333
334. Body_858_sldprt_1334
335. Body_859_sldprt_1335
336. Body_860_sldprt_1336
337. Body_861_sldprt_1337
338. Body_862_sldprt_1338
339. Body_863_sldprt_1339
340. Body_864_sldprt_1340
341. Body_865_sldprt_1341
342. Body_866_sldprt_1342
343. Body_867_sldprt_1343
344. Body_868_sldprt_1344
345. Body_869_sldprt_1345
346. Body_870_sldprt_1346
347. Body_871_sldprt_1347
348. Body_872_sldprt_1348
349. Body_873_sldprt_1349
350. Body_874_sldprt_1350
351. Body_875_sldprt_1351
352. Body_876_sldprt_1352
353. Body_877_sldprt_1353
354. Body_878_sldprt_1354
355. Body_879_sldprt_1355
356. Body_880_sldprt_1356
357. Body_881_sldprt_1357
358. Body_882_sldprt_1358
359. Body_883_sldprt_1359
360. Body_884_sldprt_1360
361. Body_885_sldprt_1361
362. Body_886_sldprt_1362
363. Body_887_sldprt_1363
364. Body_888_sldprt_1364
365. Body_889_sldprt_1365
366. Body_890_sldprt_1366
367. Body_891_sldprt_1367
368. Body_892_sldprt_1368
369. Body_893_sldprt_1369
370. Body_894_sldprt_1370
371. Body_895_sldprt_1371
372. Body_896_sldprt_1372
373. Body_897_sldprt_1373
374. Body_898_sldprt_1374
375. Body_899_sldprt_1375
376. Body_900_sldprt_1376
377. Body_901_sldprt_1377
378. Body_902_sldprt_1378
379. Body_903_sldprt_1379
380. Body_904_sldprt_1380
381. Body_905_sldprt_1381
382. Body_906_sldprt_1382
383. Body_907_sldprt_1383
384. Body_908_sldprt_1384
385. Body_909_sldprt_1385
386. Body_910_sldprt_1386
387. Body_911_sldprt_1387
388. Body_912_sldprt_1388
389. Body_913_sldprt_1389
390. Body_914_sldprt_1390
391. Body_915_sldprt_1391
392. Body_916_sldprt_1392
393. Body_917_sldprt_1393
394. Body_918_sldprt_1394
395. Body_919_sldprt_1395
396. Body_920_sldprt_1396
397. Body_921_sldprt_1397
398. Body_922_sldprt_1398
399. Body_923_sldprt_1399
400. Body_924_sldprt_1400
401. Body_925_sldprt_1401
402. Body_926_sldprt_1402
403. Body_927_sldprt_1403
404. Body_928_sldprt_1404
405. Body_929_sldprt_1405
406. Body_930_sldprt_1406
407. Body_931_sldprt_1407
408. Body_932_sldprt_1408
409. Body_933_sldprt_1409
410. Body_934_sldprt_1410
411. Body_935_sldprt_1411
412. Body_936_sldprt_1412
413. Body_937_sldprt_1413
414. Body_938_sldprt_1414
415. Body_939_sldprt_1415
416. Body_940_sldprt_1416
417. Body_941_sldprt_1417
418. Body_942_sldprt_1418
419. Body_943_sldprt_1419
420. Body_944_sldprt_1420
421. Body_945_sldprt_1421
422. Body_946_sldprt_1422
423. Body_947_sldprt_1423
424. Body_948_sldprt_1424
425. Body_949_sldprt_1425
426. Body_950_sldprt_1426
427. Body_951_sldprt_1427
428. Body_952_sldprt_1428
429. Body_953_sldprt_1429
430. Body_954_sldprt_1430
431. Body_955_sldprt_1431
432. Body_956_sldprt_1432
433. Body_957_sldprt_1433
434. Body_958_sldprt_1434
435. Body_959_sldprt_1435
436. Body_960_sldprt_1436
437. Body_961_sldprt_1437
438. Body_962_sldprt_1438
439. Body_963_sldprt_1439
440. Body_964_sldprt_1440
441. Body_965_sldprt_1441
442. Body_966_sldprt_1442
443. Body_967_sldprt_1443
444. Body_968_sldprt_1444
445. Body_969_sldprt_1445
446. Body_970_sldprt_1446
447. Body_971_sldprt_1447
448. Body_972_sldprt_1448
449. Body_973_sldprt_1449
450. Body_974_sldprt_1450
451. Body_975_sldprt_1451
452. Body_976_sldprt_1452
453. Body_977_sldprt_1453
454. Body_978_sldprt_1454
455. Body_979_sldprt_1455
456. Body_980_sldprt_1456
457. Body_981_sldprt_1457
458. Body_982_sldprt_1458
459. Body_983_sldprt_1459
460. Body_984_sldprt_1460
461. Body_985_sldprt_1461
462. Body_986_sldprt_1462
463. Body_987_sldprt_1463
464. Body_988_sldprt_1464
465. Body_989_sldprt_1465
466. Body_990_sldprt_1466
467. Body_991_sldprt_1467
468. Body_992_sldprt_1468
469. Body_993_sldprt_1469
470. Body_994_sldprt_1470
471. Body_995_sldprt_1471
472. Body_996_sldprt_1472
473. Body_997_sldprt_1473
474. Body_998_sldprt_1474
475. Body_999_sldprt_1475
476. Body_1000_sldprt_1476
477. Body_1001_sldprt_1477
478. Body_1002_sldprt_1478
479. Body_1003_sldprt_1479
480. Body_1004_sldprt_1480
481. Body_1005_sldprt_1481
482. Body_1006_sldprt_1482
483. Body_1007_sldprt_1483
484. Body_1008_sldprt_1484
485. Body_1009_sldprt_1485
486. Body_1010_sldprt_1486
487. Body_1011_sldprt_1487
488. Body_1012_sldprt_1488
489. Body_1013_sldprt_1489
490. Body_1014_sldprt_1490
491. Body_1015_sldprt_1491
492. Body_1016_sldprt_1492
493. Body_1017_sldprt_1493
494. Body_1018_sldprt_1494
495. Body_1019_sldprt_1495
496. Body_1020_sldprt_1496
497. Body_1021_sldprt_1497
498. Body_1022_sldprt_1498
499. Body_1023_sldprt_1499
500. Body_1024_sldprt_1500
501. Body_1025_sldprt_1501
502. Body_1026_sldprt_1502
503. Body_1027_sldprt_1503
504. Body_1028_sldprt_1504
505. Body_1029_sldprt_1505
506. Body_1030_sldprt_1506
507. Body_1031_sldprt_1507
508. Body_1032_sldprt_1508
509. Body_1033_sldprt_1509
510. Body_1034_sldprt_1510
511. Body_1035_sldprt_1511
512. Body_1036_sldprt_1512
513. Body_1037_sldprt_1513
514. Body_1038_sldprt_1514
515. Body_1039_sldprt_1515
516. Body_1040_sldprt_1516
517. Body_1041_sldprt_1517
518. Body_1042_sldprt_1518
519. Body_1043_sldprt_1519
520. Body_1044_sldprt_1520
521. Body_1045_sldprt_1521
522. Body_1046_sldprt_1522
523. Body_1047_sldprt_1523
524. Body_1048_sldprt_1524
525. Body_1049_sldprt_1525
526. Body_1050_sldprt_1526
527. Body_1051_sldprt_1527
528. Body_1052_sldprt_1528
529. Body_1053_sldprt_1529
530. Body_1054_sldprt_1530
531. Body_1055_sldprt_1531
532. Body_1056_sldprt_1532
533. Body_1057_sldprt_1533
534. Body_1058_sldprt_1534
535. Body_1059_sldprt_1535
536. Body_1060_sldprt_1536
537. Body_1061_sldprt_1537
538. Body_1062_sldprt_1538
539. Body_1063_sldprt_1539
540. Body_1064_sldprt_1540
541. Body_1065_sldprt_1541
542. Body_1066_sldprt_1542
543. Body_1067_sldprt_1543
544. Body_1068_sldprt_1544
545. Body_1069_sldprt_1545
546. Body_1070_sldprt_1546
547. Body_1071_sldprt_1547
548. Body_1072_sldprt_1548
549. Body_1073_sldprt_1549
550. Body_1074_sldprt_1550
551. Body_1075_sldprt_1551
552. Body_1076_sldprt_1552
553. Body_1077_sldprt_1553
554. Body_1078_sldprt_1554
555. Body_1079_sldprt_1555
556. Body_1080_sldprt_1556
557. Body_1081_sldprt_1557
558. Body_1082_sldprt_1558
559. Body_1083_sldprt_1559
560. Body_1084_sldprt_1560
561. Body_1085_sldprt_1561
562. Body_1086_sldprt_1562
563. Body_1087_sldprt_1563
564. Body_1088_sldprt_1564
565. Body_1089_sldprt_1565
566. Body_1090_sldprt_1566
567. Body_1091_sldprt_1567
568. Body_1092_sldprt_1568
569. Body_1093_sldprt_1569
570. Body_1094_sldprt_1570
571. Body_1095_sldprt_1571
572. Body_1096_sldprt_1572
573. Body_1097_sldprt_1573
574. Body_1098_sldprt_1574
575. Body_1099_sldprt_1575
576. Body_1100_sldprt_1576
577. Body_1101_sldprt_1577
578. Body_1102_sldprt_1578
579. Body_1103_sldprt_1579
580. Body_1104_sldprt_1580
581. Body_1105_sldprt_1581
582. Body_1106_sldprt_1582
583. Body_1107_sldprt_1583
584. Body_1108_sldprt_1584
585. Body_1109_sldprt_1585
586. Body_1110_sldprt_1586
587. Body_1111_sldprt_1587
588. Body_1112_sldprt_1588
589. Body_1113_sldprt_1589
590. Body_1114_sldprt_1590
591. Body_1115_sldprt_1591
592. Body_1116_sldprt_1592
593. Body_1117_sldprt_1593
594. Body_1118_sldprt_1594
595. Body_1119_sldprt_1595
596. Body_1120_sldprt_1596
597. Body_1121_sldprt_1597
598. Body_1122_sldprt_1598
599. Body_1123_sldprt_1599
600. Body_1124_sldprt_1600
601. Body_1125_sldprt_1601
602. Body_1126_sldprt_1602
603. Body_1127_sldprt_1603
604. Body_1128_sldprt_1604
605. Body_1129_sldprt_1605
606. Body_1130_sldprt_1606
607. Body_1131_sldprt_1607
608. Body_1132_sldprt_1608
609. Body_1133_sldprt_1609
610. Body_1134_sldprt_1610
611. Body_1135_sldprt_1611
612. Body_1136_sldprt_1612
613. Body_1137_sldprt_1613
614. Body_1138_sldprt_1614
615. Body_1139_sldprt_1615
616. Body_1140_sldprt_1616
617. Body_1141_sldprt_1617
618. Body_1142_sldprt_1618
619. Body_1143_sldprt_1619
620. Body_1144_sldprt_1620
621. Body_1145_sldprt_1621
622. Body_1146_sldprt_1622
623. Body_1147_sldprt_1623
624. Body_1148_sldprt_1624
625. Body_1149_sldprt_1625
626. Body_1150_sldprt_1626
627. Body_1151_sldprt_1627
628. Body_1152_sldprt_1628
629. Body_1153_sldprt_1629
630. Body_1154_sldprt_1630
631. Body_1155_sldprt_1631
632. Body_1156_sldprt_1632
633. Body_1157_sldprt_1633
634. Body_1158_sldprt_1634
635. Body_1159_sldprt_1635
636. Body_1160_sldprt_1636
637. Body_1161_sldprt_1637
638. Body_1162_sldprt_1638
639. Body_1163_sldprt_1639
640. Body_1164_sldprt_1640
641. Body_1165_sldprt_1641
642. Body_1166_sldprt_1642
643. Body_1167_sldprt_1643
644. Body_1168_sldprt_1644
645. Body_1169_sldprt_1645
646. Body_1170_sldprt_1646
647. Body_1171_sldprt_1647
648. Body_1172_sldprt_1648
649. Body_1173_sldprt_1649
650. Body_1174_sldprt_1650
651. Body_1175_sldprt_1651
652. Body_1176_sldprt_1652
653. Body_1177_sldprt_1653
654. Body_1178_sldprt_1654
655. Body_1179_sldprt_1655
656. Body_1180_sldprt_1656
657. Body_1181_sldprt_1657
658. Body_1182_sldprt_1658
659. Body_1183_sldprt_1659
660. Body_1184_sldprt_1660
661. Body_1185_sldprt_1661
662. Body_1186_sldprt_1662
663. Body_1187_sldprt_1663
664. Body_1188_sldprt_1664
665. Body_1189_sldprt_1665
666. Body_1190_sldprt_1666
667. Body_1191_sldprt_1667
668. Body_1192_sldprt_1668
669. Body_1193_sldprt_1669
670. Body_1194_sldprt_1670
671. Body_1195_sldprt_1671
672. Body_1196_sldprt_1672
673. Body_1197_sldprt_1673
674. Body_1198_sldprt_1674
675. Body_1199_sldprt_1675
676. Body_1200_sldprt_1676
677. Body_1201_sldprt_1677
678. Body_1202_sldprt_1678
679. Body_1203_sldprt_1679
680. Body_1204_sldprt_1680
681. Body_1205_sldprt_1681
682. Body_1206_sldprt_1682
683. Body_1207_sldprt_1683
684. Body_1208_sldprt_1684
685. Body_1209_sldprt_1685
686. Body_1210_sldprt_1686
687. Body_1211_sldprt_1687
688. Body_1212_sldprt_1688
689. Body_1213_sldprt_1689
690. Body_1214_sldprt_1690
691. Body_1215_sldprt_1691
692. Body_1216_sldprt_1692
693. Body_1217_sldprt_1693
694. Body_1218_sldprt_1694
695. Body_1219_sldprt_1695
696. Body_1220_sldprt_1696
697. Body_1221_sldprt_1697
698. Body_1222_sldprt_1698
699. Body_1223_sldprt_1699
700. Body_1224_sldprt_1700
701. Body_1225_sldprt_1701
702. Body_1226_sldprt_1702
703. Body_1227_sldprt_1703
704. Body_1228_sldprt_1704
705. Body_1229_sldprt_1705
706. Body_1230_sldprt_1706
707. Body_1231_sldprt_1707
708. Body_1232_sldprt_1708
709. Body_1233_sldprt_1709
710. Body_1234_sldprt_1710
711. Body_1235_sldprt_1711
712. Body_1236_sldprt_1712
713. Body_1237_sldprt_1713
714. Body_1238_sldprt_1714
715. Body_1239_sldprt_1715
716. Body_1240_sldprt_1716
717. Body_1241_sldprt_1717
718. Body_1242_sldprt_1718
719. Body_1243_sldprt_1719
720. Body_1244_sldprt_1720
721. Body_1245_sldprt_1721
722. Body_1246_sldprt_1722
723. Body_1247_sldprt_1723
724. Body_1248_sldprt_1724
725. Body_1249_sldprt_1725
726. Body_1250_sldprt_1726
727. Body_1251_sldprt_1727
728. Body_1252_sldprt_1728
729. Body_1253_sldprt_1729
730. Body_1254_sldprt_1730
731. Body_1255_sldprt_1731
732. Body_1256_sldprt_1732
733. Body_1257_sldprt_1733
734. Body_1258_sldprt_1734
735. Body_1259_sldprt_1735
736. Body_1260_sldprt_1736
737. Body_1261_sldprt_1737
738. Body_1262_sldprt_1738
739. Body_1263_sldprt_1739
740. Body_1264_sldprt_1740
741. Body_1265_sldprt_1741
742. Body_1266_sldprt_1742
743. Body_1267_sldprt_1743
744. Body_1268_sldprt_1744
745. Body_1269_sldprt_1745
746. Body_1270_sldprt_1746
747. Body_1271_sldprt_1747
748. Body_1272_sldprt_1748
749. Body_1273_sldprt_1749
750. Body_1274_sldprt_1750
751. Body_1275_sldprt_1751
752. Body_1276_sldprt_1752
753. Body_1277_sldprt_1753
754. Body_1278_sldprt_1754
755. Body_1279_sldprt_1755
756. Body_1280_sldprt_1756
757. Body_1281_sldprt_1757
758. Body_1282_sldprt_1758
759. Body_1283_sldprt_1759
760. Body_1284_sldprt_1760
761. Body_1285_sldprt_1761
762. Body_1286_sldprt_1762
763. Body_1287_sldprt_1763
764. Body_1288_sldprt_1764
765. Body_1289_sldprt_1765
766. Body_1290_sldprt_1766
767. Body_1291_sldprt_1767
768. Body_1292_sldprt_1768
769. Body_1293_sldprt_1769
770. Body_1294_sldprt_1770
771. Body_1295_sldprt_1771
772. Body_1296_sldprt_1772
773. Body_1297_sldprt_1773
774. Body_1298_sldprt_1774
775. Body_1299_sldprt_1775
776. Body_1300_sldprt_1776
777. Body_1301_sldprt_1777
778. Body_1302_sldprt_1778
779. Body_1303_sldprt_1779
780. Body_1304_sldprt_1780
781. Body_1305_sldprt_1781
782. Body_1306_sldprt_1782
783. Body_1307_sldprt_1783
784. Body_1308_sldprt_1784
785. Body_1309_sldprt_1785
786. Body_1310_sldprt_1786
787. Body_1311_sldprt_1787
788. Body_1312_sldprt_1788
789. Body_1313_sldprt_1789
790. Body_1314_sldprt_1790
791. Body_1315_sldprt_1791
792. Body_1316_sldprt_1792
793. Body_1317_sldprt_1793
794. Body_1318_sldprt_1794
795. Body_1319_sldprt_1795
796. Body_1320_sldprt_1796
797. Body_1321_sldprt_1797
798. Body_1322_sldprt_1798
799. Body_1323_sldprt_1799
800. Body_1324_sldprt_1800
801. Body_1325_sldprt_1801
802. Body_1326_sldprt_1802
803. Body_1327_sldprt_1803
804. Body_1328_sldprt_1804
805. Body_1329_sldprt_1805
806. Body_1330_sldprt_1806
807. Body_1331_sldprt_1807
808. Body_1332_sldprt_1808
809. Body_1333_sldprt_1809
810. Body_1334_sldprt_1810
811. Body_1335_sldprt_1811
812. Body_1336_sldprt_1812
813. Body_1337_sldprt_1813
814. Body_1338_sldprt_1814
815. Body_1339_sldprt_1815
816. Body_1340_sldprt_1816
817. Body_1341_sldprt_1817
818. Body_1342_sldprt_1818
819. Body_1343_sldprt_1819
820. Body_1344_sldprt_1820
821. Body_1345_sldprt_1821
822. Body_1346_sldprt_1822
823. Body_1347_sldprt_1823
824. Body_1348_sldprt_1824
825. Body_1349_sldprt_1825
826. Body_1350_sldprt_1826
827. Body_1351_sldprt_1827
828. Body_1352_sldprt_1828
829. Body_1353_sldprt_1829
830. Body_1354_sldprt_1830
831. Body_1355_sldprt_1831
832. Body_1356_sldprt_1832
833. Body_1357_sldprt_1833
834. Body_1358_sldprt_1834
835. Body_1359_sldprt_1835
836. Body_1360_sldprt_1836
837. Body_1361_sldprt_1837
838. Body_1362_sldprt_1838
839. Body_1363_sldprt_1839
840. Body_1364_sldprt_1840
841. Body_1365_sldprt_1841
842. Body_1366_sldprt_1842
843. Body_1367_sldprt_1843
844. Body_1368_sldprt_1844
845. Body_1369_sldprt_1845
846. Body_1370_sldprt_1846
847. Body_1371_sldprt_1847
848. Body_1372_sldprt_1848
849. Body_1373_sldprt_1849
850. Body_1374_sldprt_1850
851. Body_1375_sldprt_1851
852. Body_1376_sldprt_1852
853. Body_1377_sldprt_1853
854. Body_1378_sldprt_1854
855. Body_1379_sldprt_1855
856. Body_1380_sldprt_1856
857. Body_1381_sldprt_1857
858. Body_1382_sldprt_1858
859. Body_1383_sldprt_1859
860. Body_1384_sldprt_1860
861. Body_1385_sldprt_1861
862. Body_1386_sldprt_1862
863. Body_1387_sldprt_1863
864. Body_1388_sldprt_1864
865. Body_1389_sldprt_1865
866. Body_1390_sldprt_1866
867. Body_1391_sldprt_1867
868. Body_1392_sldprt_1868
869. Body_1393_sldprt_1869
870. Body_1394_sldprt_1870
871. Body_1395_sldprt_1871
872. Body_1396_sldprt_1872
873. Body_1397_sldprt_1873
874. Body_1398_sldprt_1874
875. Body_1399_sldprt_1875
876. Body_1400_sldprt_1876
877. Body_1401_sldprt_1877
878. Body_1402_sldprt_1878
879. Body_1403_sldprt_1879
880. Body_1404_sldprt_1880
881. Body_1405_sldprt_1881
882. Body_1406_sldprt_1882
883. Body_1407_sldprt_1883
884. Body_1408_sldprt_1884
885. Body_1409_sldprt_1885
886. Body_1410_sldprt_1886
887. Body_1411_sldprt_1887
888. Body_1412_sldprt_1888
889. Body_1413_sldprt_1889
890. Body_1414_sldprt_1890
891. Body_1415_sldprt_1891
892. Body_1416_sldprt_1892
893. Body_1417_sldprt_1893
894. Body_1418_sldprt_1894
895. Body_1419_sldprt_1895
896. Body_1420_sldprt_1896
897. Body_1421_sldprt_1897
898. Body_1422_sldprt_1898
899. Body_1423_sldprt_1899
900. Body_1424_sldprt_1900
901. Body_1425_sldprt_1901
902. Body_1426_sldprt_1902
903. Body_1427_sldprt_1903
904. Body_1428_sldprt_1904
905. Body_1429_sldprt_1905
906. Body_1430_sldprt_1906
907. Body_1431_sldprt_1907
908. Body_1432_sldprt_1908
909. Body_1433_sldprt_1909
910. Body_1434_sldprt_1910
911. Body_1435_sldprt_1911
912. Body_1436_sldprt_1912
913. Body_1437_sldprt_1913
914. Body_1438_sldprt_1914
915. Body_1439_sldprt_1915
916. Body_1440_sldprt_1916
917. Body_1441_sldprt_1917
918. Body_1442_sldprt_1918
919. Body_1443_sldprt_1919
920. Body_1444_sldprt_1920
921. Body_1445_sldprt_1921
922. Body_1446_sldprt_1922
923. Body_1447_sldprt_1923
924. Body_1448_sldprt_1924
925. Body_1449_sldprt_1925
926. Body_1450_sldprt_1926
927. Body_1451_sldprt_1927
928. Body_1452_sldprt_1928
929. Body_1453_sldprt_1929
930. Body_1454_sldprt_1930
931. Body_1455_sldprt_1931
932. Body_1456_sldprt_1932
933. Body_1457_sldprt_1933
934. Body_1458_sldprt_1934
935. Body_1459_sldprt_1935
936. Body_1460_sldprt_1936
937. Body_1461_sldprt_1937
938. Body_1462_sldprt_1938
939. Body_1463_sldprt_1939
940. Body_1464_sldprt_1940
941. Body_1465_sldprt_1941
942. Body_1466_sldprt_1942
